# Autodesk Inventor assembly: Head
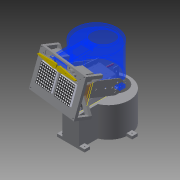
[picture p0: Inventor's stored thumbnail of the model, 180x180]
Saved by Autodesk Inventor 2015 (Build 190159000, 159)
## iProperties
Created: 2015-03-10
Part Number: Head
Document SubType Name: Assembly
Designer: ChristopherEvan
Author: ChristopherEvan
## Documents named in this file (8)
- C:\Users\ChristopherEvan\Documents\Inventor\MAKE\Head\Head.iam
- C:\Users\ChristopherEvan\Documents\Inventor\MAKE\Pan_Tilt\Pan_Tilt.iam
- C:\Users\ChristopherEvan\Documents\Inventor\MAKE\Enclosure\LCD\Face.ipt
- C:\Users\ChristopherEvan\Documents\Inventor\MAKE\Head\Eyes\led_matrix.ipt
- C:\Users\ChristopherEvan\Documents\Inventor\MAKE\Enclosure\LCD\Face3.ipt
- C:\Users\ChristopherEvan\Documents\Inventor\MAKE\Head\Eyebrows\Servo\MicroServo9g.iam
- C:\Users\ChristopherEvan\Documents\Inventor\MAKE\Enclosure\LCD\Eyebrows.ipt
- C:\Users\ChristopherEvan\Documents\Inventor\MAKE\Neck.ipt
## Components (9 placed, 7 different names)
1. Pan_Tilt:1 [sub-assembly] — Flush:2, Flush:5, Flush:6
2. Face:1 — Flush:2, Flush:3
3. led_matrix:1 — Mate:1, Mate:2, Mate:3
4. Face3:1 — Flush:3, Mate:1, Mate:2, Mate:3, Mate:4, Mate:5, Mate:6, Mate:7, Mate:10, Angle:1, Angle:2, Mate:11, Mate:12, Mate:13, Mate:14
5. led_matrix:2 — Mate:4, Mate:5, Mate:6
6. MicroServo9g:1 [sub-assembly] — Mate:7, Angle:1, Mate:11, Mate:12, Flush:4
7. MicroServo9g:2 [sub-assembly] — Mate:10, Angle:2, Mate:13, Mate:14
8. Eyebrows:1 — Flush:4
9. Neck:1 — Flush:5, Flush:6
## Relationships (19: Mate 12, Flush 5, Angle 2)
- Flush:2: Pan_Tilt:1 ↔ Face:1
- Flush:3: Face:1 ↔ Face3:1
- Mate:1: led_matrix:1 ↔ Face3:1
- Mate:2: led_matrix:1 ↔ Face3:1
- Mate:3: led_matrix:1 ↔ Face3:1
- Mate:4: Face3:1 ↔ led_matrix:2
- Mate:5: Face3:1 ↔ led_matrix:2
- Mate:6: Face3:1 ↔ led_matrix:2
- Mate:7: Face3:1 ↔ MicroServo9g:1
- Mate:10: Face3:1 ↔ MicroServo9g:2
- Angle:1 (0 deg): Face3:1 ↔ MicroServo9g:1
- Angle:2 (0 deg): Face3:1 ↔ MicroServo9g:2
- Mate:11: Face3:1 ↔ MicroServo9g:1
- Mate:12: Face3:1 ↔ MicroServo9g:1
- Mate:13: Face3:1 ↔ MicroServo9g:2
- Mate:14: Face3:1 ↔ MicroServo9g:2
- Flush:4: MicroServo9g:1 ↔ Eyebrows:1
- Flush:5: Pan_Tilt:1 ↔ Neck:1
- Flush:6: Pan_Tilt:1 ↔ Neck:1
